# Autodesk Inventor assembly: CL1-200
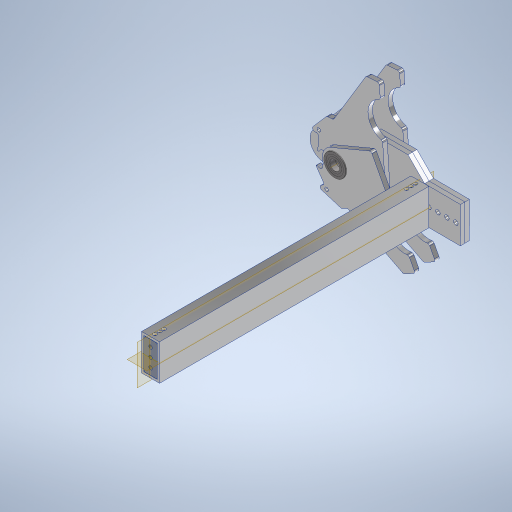
[picture p0: Inventor's stored thumbnail of the model, 512x512]
Saved by Autodesk Inventor 2023.4 (Build 274418000, 418)
## iProperties
Created: 2025-01-18
Part Number: CL1-200
Document SubType Name: Assembly
Designer: mavericks
Author: mavericks
## Documents named in this file (6)
- C:\Users\mavericks\Documents\Robotics\GitHub\2025-ReefScape---CAD\Climber\CL1-200.iam
- C:\Users\mavericks\Documents\Robotics\GitHub\2025-ReefScape---CAD\Climber\Cl1-100.iam
- C:\Users\mavericks\Documents\Robotics\GitHub\2025-ReefScape---CAD\Climber\CL1-002.ipt
- C:\Users\mavericks\Documents\Robotics\GitHub\2025-ReefScape---CAD\Climber\CL1-001.ipt
- C:\Users\mavericks\Documents\Robotics\GitHub\2025-ReefScape---CAD\COMMON PARTS\BEARINGS\13_75mm_1_2_ThunderHex_ID_x_1_125_OD_x_0_313_WD_Flanged_Bearing_217-4006_MIR.ipt
- C:\Users\mavericks\Documents\Robotics\GitHub\2025-ReefScape---CAD\Climber\CL1-006.ipt
## Components (13 placed, 5 different names)
1. Cl1-100:1 [sub-assembly] — Insert:1, Insert:2
2. CL1-002:1 — Mate:2, Mate:3, Mate:17, Flush:4, Insert:4
3. CL1-002:2 — Mate:4, Mate:9, Mate:13, Flush:4
4. CL1-002:3 — Mate:6, Mate:7, Mate:13, Flush:3, Insert:3
5. CL1-002:4 — Mate:5, Mate:8, Mate:17, Flush:3
6. CL1-001:1 — Mate:1, Flush:1, Flush:2, Insert:1, Insert:2, Mate:14, Mate:15
7. CL1-001:2 — Mate:1, Flush:1, Flush:2, Mate:10, Mate:11
8. 13_75mm_1_2_ThunderHex_ID_x_1_125_OD_x_0_313_WD_Flanged_Bearing_217-4006_MIR:1 — Mate:4, Mate:9, Mate:10, Mate:11, Mate:12
9. 13_75mm_1_2_ThunderHex_ID_x_1_125_OD_x_0_313_WD_Flanged_Bearing_217-4006_MIR:2 — Mate:2, Mate:3, Mate:16
10. 13_75mm_1_2_ThunderHex_ID_x_1_125_OD_x_0_313_WD_Flanged_Bearing_217-4006_MIR:3 — Mate:6, Mate:7, Mate:12
11. 13_75mm_1_2_ThunderHex_ID_x_1_125_OD_x_0_313_WD_Flanged_Bearing_217-4006_MIR:4 — Mate:5, Mate:8, Mate:14, Mate:15, Mate:16
12. CL1-006:1 — Insert:3
13. CL1-006:2 — Insert:4
## Relationships (25: Mate 17, Flush 4, Insert 4)
- Mate:1: CL1-001:1 ↔ CL1-001:2
- Flush:1: CL1-001:1 ↔ CL1-001:2
- Flush:2: CL1-001:1 ↔ CL1-001:2
- Insert:1: Cl1-100:1 ↔ CL1-001:1
- Insert:2: Cl1-100:1 ↔ CL1-001:1
- Mate:2: CL1-002:1 ↔ 13_75mm_1_2_ThunderHex_ID_x_1_125_OD_x_0_313_WD_Flanged_Bearing_217-4006_MIR:2
- Mate:3: CL1-002:1 ↔ 13_75mm_1_2_ThunderHex_ID_x_1_125_OD_x_0_313_WD_Flanged_Bearing_217-4006_MIR:2
- Mate:4: CL1-002:2 ↔ 13_75mm_1_2_ThunderHex_ID_x_1_125_OD_x_0_313_WD_Flanged_Bearing_217-4006_MIR:1
- Mate:5: CL1-002:4 ↔ 13_75mm_1_2_ThunderHex_ID_x_1_125_OD_x_0_313_WD_Flanged_Bearing_217-4006_MIR:4
- Mate:6: CL1-002:3 ↔ 13_75mm_1_2_ThunderHex_ID_x_1_125_OD_x_0_313_WD_Flanged_Bearing_217-4006_MIR:3
- Mate:7: CL1-002:3 ↔ 13_75mm_1_2_ThunderHex_ID_x_1_125_OD_x_0_313_WD_Flanged_Bearing_217-4006_MIR:3
- Mate:8: CL1-002:4 ↔ 13_75mm_1_2_ThunderHex_ID_x_1_125_OD_x_0_313_WD_Flanged_Bearing_217-4006_MIR:4
- Mate:9: CL1-002:2 ↔ 13_75mm_1_2_ThunderHex_ID_x_1_125_OD_x_0_313_WD_Flanged_Bearing_217-4006_MIR:1
- Mate:10: CL1-001:2 ↔ 13_75mm_1_2_ThunderHex_ID_x_1_125_OD_x_0_313_WD_Flanged_Bearing_217-4006_MIR:1
- Mate:11: CL1-001:2 ↔ 13_75mm_1_2_ThunderHex_ID_x_1_125_OD_x_0_313_WD_Flanged_Bearing_217-4006_MIR:1
- Mate:12: 13_75mm_1_2_ThunderHex_ID_x_1_125_OD_x_0_313_WD_Flanged_Bearing_217-4006_MIR:1 ↔ 13_75mm_1_2_ThunderHex_ID_x_1_125_OD_x_0_313_WD_Flanged_Bearing_217-4006_MIR:3
- Mate:13: CL1-002:2 ↔ CL1-002:3
- Mate:14: CL1-001:1 ↔ 13_75mm_1_2_ThunderHex_ID_x_1_125_OD_x_0_313_WD_Flanged_Bearing_217-4006_MIR:4
- Mate:15: CL1-001:1 ↔ 13_75mm_1_2_ThunderHex_ID_x_1_125_OD_x_0_313_WD_Flanged_Bearing_217-4006_MIR:4
- Mate:16: 13_75mm_1_2_ThunderHex_ID_x_1_125_OD_x_0_313_WD_Flanged_Bearing_217-4006_MIR:2 ↔ 13_75mm_1_2_ThunderHex_ID_x_1_125_OD_x_0_313_WD_Flanged_Bearing_217-4006_MIR:4
- Mate:17: CL1-002:1 ↔ CL1-002:4
- Flush:3: CL1-002:3 ↔ CL1-002:4
- Flush:4: CL1-002:1 ↔ CL1-002:2
- Insert:3: CL1-002:3 ↔ CL1-006:1
- Insert:4: CL1-002:1 ↔ CL1-006:2
